# Autodesk Inventor assembly: MotorAssemblyV4
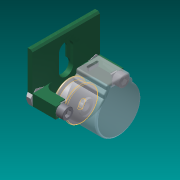
[picture p0: Inventor's stored thumbnail of the model, 180x180]
Saved by Autodesk Inventor 2013 (Build 170138000, 138)
## iProperties
Created: 2013-08-18
Part Number: MotorAssemblyV4
Document SubType Name: Assembly
Designer: Sawaiz
Author: Sawaiz
## Documents named in this file (5)
- S:\Sawaiz\Documents\3D Modeling\Inventor\PolarGraph\MotorAssemblyV4.iam
- S:\Sawaiz\Documents\3D Modeling\Inventor\PolarGraph\MotorClipV4.ipt
- S:\Sawaiz\Documents\3D Modeling\Inventor\PolarGraph\MonoFilamentSpool22mm.iam
- S:\Sawaiz\Documents\3D Modeling\Inventor\PolarGraph\Imported Components\91841A009\91841A009.ipt
- S:\Sawaiz\Documents\3D Modeling\Inventor\Content Center Files\R2013\en-US\ANSI B18.3(05)\ANSI B18.3 - 8-32 UNC - 0.625(31).ipt
## Components (6 placed, 4 different names)
1. MotorClipV4:1 — Mate:1, Mate:2, Mate:3, Mate:4, Mate:5, Mate:6, Mate:7, Flush:2, Flush:3, Mate:9, Mate:10
2. MonoFilamentSpool22mm:1 [sub-assembly] — Mate:1, Mate:2, Mate:3, Flush:1, Mate:8
3. 91841A009:1 — Mate:5, Flush:3, Mate:9
4. 91841A009:2 — Mate:4, Flush:2, Mate:10
5. Hexagon Socket Head Cap Screw - Inch No. 8 - 32 UNC - 5/8:1 — Mate:7, Mate:8
6. Hexagon Socket Head Cap Screw - Inch No. 8 - 32 UNC - 5/8:2 — Mate:6, Flush:1
## Relationships (13: Mate 10, Flush 3)
- Mate:1: MotorClipV4:1 ↔ MonoFilamentSpool22mm:1
- Mate:2: MotorClipV4:1 ↔ MonoFilamentSpool22mm:1
- Mate:3 (0.5 mm): MotorClipV4:1 ↔ MonoFilamentSpool22mm:1
- Mate:4: MotorClipV4:1 ↔ 91841A009:2
- Mate:5: MotorClipV4:1 ↔ 91841A009:1
- Mate:6: MotorClipV4:1 ↔ Hexagon Socket Head Cap Screw - Inch No. 8 - 32 UNC - 5/8:2
- Mate:7: MotorClipV4:1 ↔ Hexagon Socket Head Cap Screw - Inch No. 8 - 32 UNC - 5/8:1
- Flush:1: MonoFilamentSpool22mm:1 ↔ Hexagon Socket Head Cap Screw - Inch No. 8 - 32 UNC - 5/8:2
- Mate:8: MonoFilamentSpool22mm:1 ↔ Hexagon Socket Head Cap Screw - Inch No. 8 - 32 UNC - 5/8:1
- Flush:2: MotorClipV4:1 ↔ 91841A009:2
- Flush:3: MotorClipV4:1 ↔ 91841A009:1
- Mate:9: MotorClipV4:1 ↔ 91841A009:1
- Mate:10: MotorClipV4:1 ↔ 91841A009:2
